# Autodesk Inventor assembly: rev4
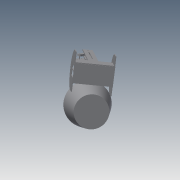
[picture p0: Inventor's stored thumbnail of the model, 180x180]
Saved by Autodesk Inventor 2015 (Build 190159000, 159)
## iProperties
Created: 2014-07-15
Part Number: rev4
Document SubType Name: Assembly
Designer: shohei
Author: shohei
## Documents named in this file (20)
- C:\Users\shohei\Documents\Inventor\FufuPounder\rev5.iam
- C:\Users\shohei\Documents\Inventor\FufuPounderLeverType\Part1.ipt
- C:\Users\shohei\Documents\Inventor\FufuPounderLeverType\Part2.ipt
- C:\Users\shohei\Documents\Inventor\FufuPounderLeverType\Part4.ipt
- C:\Users\shohei\Documents\Inventor\FufuPounderLeverType\baseboard.ipt
- C:\Users\shohei\Documents\Inventor\FufuPounderLeverType\shaft2.ipt
- C:\Users\shohei\Documents\Inventor\FufuPounderLeverType\shaft3.ipt
- C:\Users\shohei\Documents\Inventor\FufuPounderLeverType\mortar2.ipt
- C:\Users\shohei\Documents\Inventor\FufuPounderLeverType\small_lever.ipt
- C:\Users\shohei\Documents\Inventor\FufuPounderLeverType\beam.ipt
- C:\Users\shohei\Documents\Inventor\FufuPounderLeverType\shaft4.ipt
- C:\Users\shohei\Documents\Inventor\FufuPounderLeverType\block.ipt
- C:\Users\shohei\Documents\Inventor\FufuPounderLeverType\malllet2.ipt
- C:\Users\shohei\Documents\Inventor\FufuPounderLeverType\mallet_side.ipt
- C:\Users\shohei\Documents\Inventor\FufuPounder\rev5\AIP\FEA\b5sdei5mo.fins
- C:\Users\shohei\Documents\Inventor\FufuPounder\rev5\AIP\FEA\b5sdei5mo.fsat
- C:\Users\shohei\Documents\Inventor\FufuPounder\rev5\AIP\FEA\b5sdei5mo.ftes
- C:\Users\shohei\Documents\Inventor\FufuPounder\rev5\AIP\FEA\b5sdei5mo.fwiz
- C:\Users\shohei\Documents\Inventor\FufuPounder\rev5\AIP\FEA\b5sdei5pc.fmsh
- C:\Users\shohei\Documents\Inventor\FufuPounder\rev5\AIP\FEA\b5sdei5pd.fres
## Components (19 placed, 13 different names)
1. Part1:1 — Flush:15, Mate:7, Flush:23, Slider:3
2. Part1:2 — Flush:15, Flush:16, Flush:19, Mate:3, Flush:20, Mate:5, Flush:22
3. Part4:2 — Rotational:14, Cylindrical:21
4. Part2:3 — Rotational:13, Rotational:14
5. baseboard:1 — Flush:16, Mate:6, Mate:7, Mate:8, Flush:29
6. shaft2:1 — Cylindrical:21
7. mortar2:1 — Angle:3, Flush:29
8. small_lever:1 — Rotational:12, Rotational:13
9. beam:1 — Flush:19, Mate:3
10. beam:2 — Flush:20, Mate:5
11. shaft3:1 — Rigid:1
12. Part1:3 — Rigid:1, Mate:6, Flush:22, Rotational:12
13. Part1:4 — Flush:23, Mate:8, Slider:2
14. shaft4:1 — Rotational:9, Slider:2
15. block:1 — Rotational:9, Mate:9, Flush:24, Flush:25, Mate:10, Flush:26, Flush:27
16. block:2 — Slider:3
17. malllet2:1 — Angle:3
18. mallet_side:1 — Mate:10, Flush:26, Flush:27
19. mallet_side:2 — Mate:9, Flush:24, Flush:25
## Relationships (27: Flush 11, Mate 7, RevoluteJoint 4, TranslationJoint 2, WeldJoint 1, Angle 1, CylindricalJoint 1)
- Flush:15: Part1:1 ↔ Part1:2
- Flush:16: Part1:2 ↔ baseboard:1
- Flush:19: Part1:2 ↔ beam:1
- Mate:3: Part1:2 ↔ beam:1
- Flush:20: Part1:2 ↔ beam:2
- Mate:5: Part1:2 ↔ beam:2
- Rigid:1 [WeldJoint]: shaft3:1 ↔ Part1:3
- Mate:6: baseboard:1 ↔ Part1:3
- Flush:22: Part1:2 ↔ Part1:3
- Mate:7: Part1:1 ↔ baseboard:1
- Flush:23: Part1:1 ↔ Part1:4
- Mate:8: baseboard:1 ↔ Part1:4
- Rotational:9 [RevoluteJoint]: shaft4:1 ↔ block:1
- Slider:2 [TranslationJoint]: Part1:4 ↔ shaft4:1
- Angle:3 (0 deg): mortar2:1 ↔ malllet2:1
- Mate:9: block:1 ↔ mallet_side:2
- Flush:24: block:1 ↔ mallet_side:2
- Flush:25: block:1 ↔ mallet_side:2
- Mate:10: block:1 ↔ mallet_side:1
- Flush:26: block:1 ↔ mallet_side:1
- Flush:27: block:1 ↔ mallet_side:1
- Flush:29: baseboard:1 ↔ mortar2:1
- Rotational:12 [RevoluteJoint] (-5 mm): small_lever:1 ↔ Part1:3
- Rotational:13 [RevoluteJoint]: Part2:3 ↔ small_lever:1
- Rotational:14 [RevoluteJoint]: Part4:2 ↔ Part2:3
- Cylindrical:21: Part4:2 ↔ shaft2:1
- Slider:3 [TranslationJoint]: Part1:1 ↔ block:2
## Named parameters: sa_0 = -9796.95, sa_1 = -273.553, sa_2 = -1986.17
note: some values were not read from the file. Shown as the stored number, unit unknown: "sa_0", "sa_1", "sa_2".
